# Autodesk Inventor assembly: Front Cowling
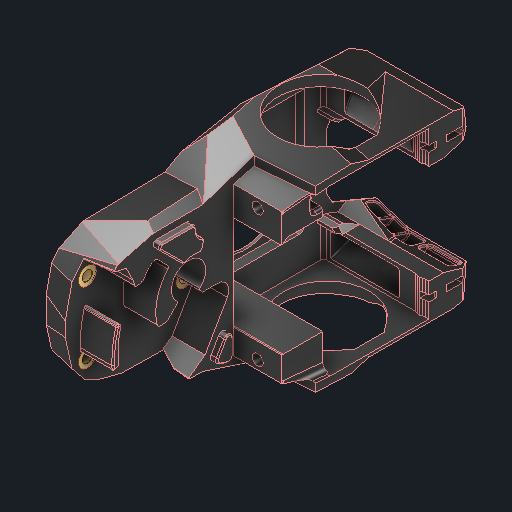
[picture p0: Inventor's stored thumbnail of the model, 512x512]
Saved by Autodesk Inventor 2025.1 (Build 291241020, 241B)
## iProperties
Created: 2025-05-09
Part Number: Front Cowling
Document SubType Name: Assembly
Designer: AdminForWorker
Title: Front Cowling
Author: AdminForWorker
## Documents named in this file (5)
- C:\Users\Joshua Eah\Documents\Voron 0.2\CAD\Master Assembly\Toolhead\Subassemblies\Front Cowling.iam
- C:\Users\Joshua Eah\Documents\Voron 0.2\CAD\Master Assembly\Toolhead\Parts\Front Cowling.ipt
- Front Cowling.ipt
- C:\Users\Joshua Eah\Documents\Voron 0.2\CAD\Master Assembly\Toolhead\Parts\Logo Insert.ipt
- C:\Users\Joshua Eah\Documents\Voron 0.2\CAD\Master Assembly\Hardware\M3 Threaded Insert.ipt
## Components (5 placed, 3 different names)
1. Front Cowling (1):1 — Insert:1, Insert:2, Insert:3
2. Logo Insert (1):1
3. M3 Threaded Insert:1 — Insert:3
4. M3 Threaded Insert:3 — Insert:1
5. M3 Threaded Insert:2 — Insert:2
## Relationships (3: Insert 3)
- Insert:1: Front Cowling (1):1 ↔ M3 Threaded Insert:3
- Insert:2: Front Cowling (1):1 ↔ M3 Threaded Insert:2
- Insert:3: Front Cowling (1):1 ↔ M3 Threaded Insert:1
